# Autodesk Inventor assembly: curve+flat
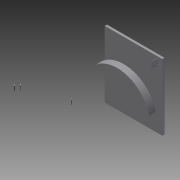
[picture p0: Inventor's stored thumbnail of the model, 180x180]
Saved by Autodesk Inventor 2011 SP1 (Build 150282100, 282)
## iProperties
Created: 2013-01-18
Part Number: curve+flat
Document SubType Name: Assembly
Designer: wes
Author: wes
## Documents named in this file (5)
- F:\ALL FILES\My Documents\GitHub\2013CAD\2013 robot\CurvedShooter\Common Chassis Parts\curve+flat.iam
- F:\ALL FILES\My Documents\GitHub\2013CAD\2013 robot\CurvedShooter\ajustableBase w mounting holes.ipt
- F:\ALL FILES\My Documents\GitHub\2013CAD\2013 robot\CurvedShooter\curvedTrack 123.47 degrees.ipt
- F:\ALL FILES\My Documents\GitHub\2013CAD\2013 robot\CurvedShooter\curveBracket.ipt
- F:\ALL FILES\My Documents\GitHub\2013CAD\2013 robot\CurvedShooter\Common Chassis Parts\.25 diameter 2'' bolt.ipt
## Components (10 placed, 4 different names)
1. ajustableBase w mounting holes:1 — Tangent:1, Insert:5, Insert:6
2. curvedTrack 123.47 degrees:1 — Tangent:1
3. curveBracket:1 — Insert:1, Insert:2, Insert:3, Insert:4
4. .25 diameter 2'' bolt:1 — Insert:4, Insert:6
5. .25 diameter 2'' bolt:2 — Insert:3
6. .25 diameter 2'' bolt:3 — Insert:2
7. .25 diameter 2'' bolt:4 — Insert:1, Insert:5
8. .25 diameter 2'' bolt:5
9. .25 diameter 2'' bolt:6
10. .25 diameter 2'' bolt:7
## Relationships (7: Insert 6, Tangent 1)
- Tangent:1: ajustableBase w mounting holes:1 ↔ curvedTrack 123.47 degrees:1
- Insert:1: curveBracket:1 ↔ .25 diameter 2'' bolt:4
- Insert:2: curveBracket:1 ↔ .25 diameter 2'' bolt:3
- Insert:3: curveBracket:1 ↔ .25 diameter 2'' bolt:2
- Insert:4: curveBracket:1 ↔ .25 diameter 2'' bolt:1
- Insert:5: ajustableBase w mounting holes:1 ↔ .25 diameter 2'' bolt:4
- Insert:6: ajustableBase w mounting holes:1 ↔ .25 diameter 2'' bolt:1
